# Autodesk Inventor assembly: spring
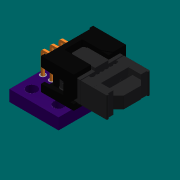
[picture p0: Inventor's stored thumbnail of the model, 180x180]
Saved by Autodesk Inventor 2016 (Build 200138000, 138)
## iProperties
Created: 2016-09-05
Part Number: spring
Document SubType Name: Assembly
Designer: sawaiz
Author: sawaiz
## Documents named in this file (6)
- C:\Users\sawaiz\oneDrive\projects\splitFlapDisplay\electronics\cad\spring\spring.iam
- C:\Users\sawaiz\oneDrive\projects\splitFlapDisplay\electronics\cad\spring\spring.ipt
- C:\Users\sawaiz\oneDrive\projects\splitFlapDisplay\electronics\cad\spring\spacer.ipt
- C:\Users\sawaiz\oneDrive\projects\splitFlapDisplay\electronics\cad\component\Preci-Dip 811\1 by 4.iam
- C:\Users\sawaiz\oneDrive\projects\splitFlapDisplay\electronics\cad\component\75867131lf\75867131lf.iam
- C:\Users\sawaiz\oneDrive\projects\splitFlapDisplay\electronics\cad\component\61200623021.ipt
## Components (5 placed, 5 different names)
1. spring:1 — Mate:1, Mate:2, Mate:3, Mate:4, Angle:1, Tangent:1, Angle:2
2. spacer:1 — Mate:1, Mate:2, Mate:3
3. 1 by 4:1 [sub-assembly] — Mate:4, Angle:1
4. 75867131lf:1 [sub-assembly] — Tangent:1, Angle:2, Mate:5, Mate:6
5. 61200623021:1 — Mate:5, Mate:6
## Relationships (9: Mate 6, Angle 2, Tangent 1)
- Mate:1: spring:1 ↔ spacer:1
- Mate:2: spring:1 ↔ spacer:1
- Mate:3: spring:1 ↔ spacer:1
- Mate:4 (0.5 mm): spring:1 ↔ 1 by 4:1
- Angle:1 (0 deg): spring:1 ↔ 1 by 4:1
- Tangent:1: spring:1 ↔ 75867131lf:1
- Angle:2 (0 deg): spring:1 ↔ 75867131lf:1
- Mate:5: 75867131lf:1 ↔ 61200623021:1
- Mate:6: 75867131lf:1 ↔ 61200623021:1
